# Autodesk Inventor assembly: Lifting Mechanism
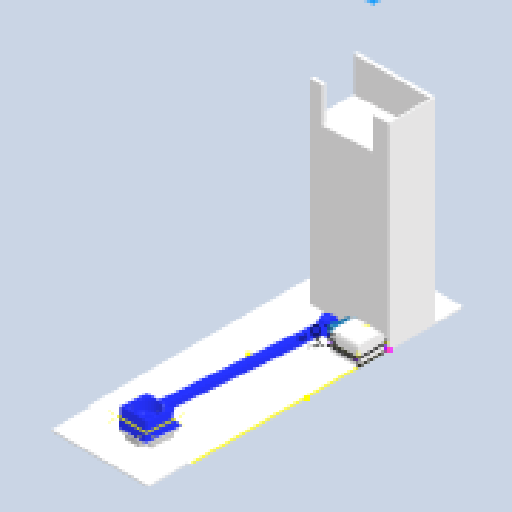
[picture p0: Inventor's stored thumbnail of the model, 512x512]
Saved by Autodesk Inventor 2025.4 (Build 294407000, 407)
## iProperties
Created: 2026-03-10
Part Number: Lifting Mechanism
Document SubType Name: Assembly
Designer: user
Author: user
## Documents named in this file (6)
- D:\basics project\Lifting Mechanism (Final)\Lifting Mechanism\Lifting Mechanism.iam
- D:\basics project\Lifting Mechanism (Final)\Lifting Mechanism\lifting base.ipt
- D:\basics project\Lifting Mechanism (Final)\Lifting Mechanism\SERVO.ipt
- D:\basics project\Lifting Mechanism (Final)\Lifting Mechanism\arm.ipt
- D:\basics project\Lifting Mechanism (Final)\Lifting Mechanism\final sensor housing.ipt
- D:\basics project\Lifting Mechanism (Final)\Lifting Mechanism\IR Module.ipt
## Components (5 placed, 5 different names)
1. lifting base:1 — Mate:1, Mate:2, Mate:5
2. SERVO:1 — Mate:1, Mate:2, Mate:5, Mate:6, Mate:7
3. arm:2 — Mate:6, Mate:7, Mate:11, Mate:12, Mate:13, Mate:14, Mate:15
4. final sensor housing:1 — Mate:8, Mate:9, Mate:10, Mate:11, Mate:12, Mate:13, Mate:14, Mate:15
5. IR Module:1 — Mate:8, Mate:9, Mate:10
## Relationships (13: Mate 13)
- Mate:1: lifting base:1 ↔ SERVO:1
- Mate:2: lifting base:1 ↔ SERVO:1
- Mate:5: lifting base:1 ↔ SERVO:1
- Mate:6: SERVO:1 ↔ arm:2
- Mate:7: SERVO:1 ↔ arm:2
- Mate:8: final sensor housing:1 ↔ IR Module:1
- Mate:9: final sensor housing:1 ↔ IR Module:1
- Mate:10: final sensor housing:1 ↔ IR Module:1
- Mate:11: arm:2 ↔ final sensor housing:1
- Mate:12: arm:2 ↔ final sensor housing:1
- Mate:13: arm:2 ↔ final sensor housing:1
- Mate:14: arm:2 ↔ final sensor housing:1
- Mate:15: arm:2 ↔ final sensor housing:1
## Named parameters: Finish1_Area = 13.1132
note: some values were not read from the file. Shown as the stored number, unit unknown: "Finish1_Area".
